# Autodesk Inventor assembly: main
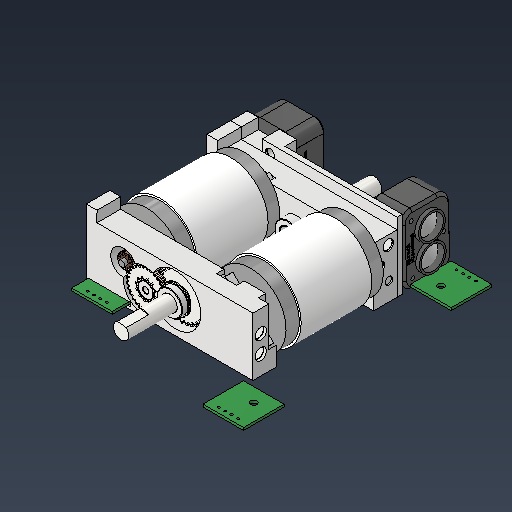
[picture p0: Inventor's stored thumbnail of the model, 512x512]
Saved by Autodesk Inventor 2026.2 (Build 302298010, 298A)
## iProperties
Created: 2026-03-09
Part Number: main
Document SubType Name: Assembly
Designer: szymo
Mass: 365.671 g
Surface Area: 1150.88 cm^2
Volume: 157.658 cm^3
Density: 2.31939 g/cm^3
Author: szymo
## Documents named in this file (18)
- D:\tech\robotyka\robots\evangelion-turbo\inventor-project\main.iam
- D:\tech\robotyka\robots\evangelion-turbo\inventor-project\drive-train.iam
- D:\tech\robotyka\robots\evangelion-turbo\inventor-project\LUNA.ipt
- D:\tech\robotyka\robots\evangelion-turbo\inventor-project\3s450mah.ipt
- D:\tech\robotyka\robots\evangelion-turbo\inventor-project\KTIR-Board.ipt
- D:\tech\robotyka\robots\evangelion-turbo\inventor-project\plug.ipt
- D:\tech\robotyka\robots\evangelion-turbo\inventor-project\FonrtMount.ipt
- D:\tech\robotyka\robots\evangelion-turbo\inventor-project\PCB_interface.ipt
- D:\tech\robotyka\robots\evangelion-turbo\inventor-project\0.96 oled\0.96 oled\0.96 oled.ipt
- D:\tech\robotyka\robots\evangelion-turbo\inventor-project\THMU 13 (SMD JOYSTICK)\THMU 13 (SMD JOYSTICK)\THMU 13 (SMD JOYSTICK).ipt
- D:\tech\robotyka\robots\evangelion-turbo\inventor-project\PCB_Controller.ipt
- D:\tech\robotyka\robots\evangelion-turbo\inventor-project\PCB_Holder_Floor.ipt
- D:\tech\robotyka\robots\evangelion-turbo\inventor-project\SteelFront.ipt
- D:\tech\robotyka\robots\evangelion-turbo\inventor-project\Ceiling.ipt
- D:\tech\robotyka\robots\evangelion-turbo\inventor-project\SpringSteelFront.ipt
- D:\tech\robotyka\robots\evangelion-turbo\inventor-project\LeftGearbox.ipt
- D:\tech\robotyka\robots\evangelion-turbo\inventor-project\LeftGearboxCoverr.ipt
- D:\tech\robotyka\robots\evangelion-turbo\inventor-project\RightGearbox.ipt
## Components (24 placed, 17 different names)
1. drive-train:1 [sub-assembly] — Flush:2, Flush:3, Flush:4, Mate:2, Mate:3, Tangent:1, Mate:18
2. 3s450mah:1 — Flush:8, Tangent:1, Flush:9
3. Ceiling:1 — Flush:64
4. LUNA:2 — Mate:1, Mate:3, Angle:2, Mate:11
5. LUNA:1 — Flush:5, Mate:2, Angle:1, Mate:12
6. LUNA:3 — Flush:22, Flush:23, Mate:6
7. LUNA:4 — Flush:24, Flush:25, Mate:7
8. KTIR-Board:1 — Flush:10, Flush:11, Flush:13
9. KTIR-Board:2 — Mate:4, Flush:12, Flush:14
10. KTIR-Board:4 — Flush:17, Flush:27, Mate:6, Mate:18
11. KTIR-Board:5 — Flush:28, Flush:29, Mate:7, Mate:19
12. SpringSteelFront:1 — Flush:65, Mate:21, Mate:22
13. SteelFront:1 — Flush:62
14. plug:1 — Mate:10, Flush:45, Mate:20
15. FonrtMount:1 — Flush:47
16. PCB_Holder_Floor:1 — Mate:25, Mate:26, Mate:27, Mate:28
17. PCB_Controller:1 — Mate:25, Mate:26
18. PCB_Controller:3 — Mate:27, Mate:28
19. LeftGearbox:1 — Flush:67
20. LeftGearboxCoverr:1 — Flush:69
21. RightGearbox:1 — Flush:71
22. PCB_interface:1 — Mate:14
23. THMU 13 (SMD JOYSTICK):1
24. 0.96 oled:1 — Mate:14
## Relationships (54: Flush 32, Mate 19, Angle 2, Tangent 1)
- Flush:2: drive-train:1
- Flush:3 (-19.2 mm): drive-train:1
- Flush:4: drive-train:1
- Flush:5 (49.5 mm): LUNA:1
- Mate:1 (-49.5 mm): LUNA:2
- Mate:2 (19 mm): drive-train:1 ↔ LUNA:1
- Mate:3 (19 mm): drive-train:1 ↔ LUNA:2
- Angle:1 (-2 deg): LUNA:1
- Angle:2 (182 deg): LUNA:2
- Flush:8 (4.5 mm): 3s450mah:1
- Tangent:1: drive-train:1 ↔ 3s450mah:1
- Flush:9 (-31.5 mm): 3s450mah:1
- Flush:10 (-49 mm): KTIR-Board:1
- Mate:4 (-49 mm): KTIR-Board:2
- Flush:11 (0.13 mm): KTIR-Board:1
- Flush:12 (0.13 mm): KTIR-Board:2
- Flush:13 (66.673 mm): KTIR-Board:1
- Flush:14 (-66.673 mm): KTIR-Board:2
- Flush:17: KTIR-Board:4
- Flush:22: LUNA:3
- Flush:23 (1 mm): LUNA:3
- Flush:24 (1 mm): LUNA:4
- Flush:25: LUNA:4
- Flush:27 (1 mm): KTIR-Board:4
- Flush:28 (1 mm): KTIR-Board:5
- Flush:29: KTIR-Board:5
- Mate:6: LUNA:3 ↔ KTIR-Board:4
- Mate:7: LUNA:4 ↔ KTIR-Board:5
- Mate:10: plug:1
- Flush:45: plug:1
- Mate:11: LUNA:2
- Mate:12: LUNA:1
- Flush:47: FonrtMount:1
- Flush:53 (-29 mm)
- Mate:14: PCB_interface:1 ↔ 0.96 oled:1
- Mate:18: drive-train:1 ↔ KTIR-Board:4
- Mate:19 (19.2 mm): KTIR-Board:5
- Flush:62: SteelFront:1
- Flush:64: Ceiling:1
- Mate:20 (-95.5 mm): plug:1
- Flush:65: SpringSteelFront:1
- Mate:21: SpringSteelFront:1
- Mate:22: SpringSteelFront:1
- Mate:25: PCB_Holder_Floor:1 ↔ PCB_Controller:1
- Mate:26: PCB_Holder_Floor:1 ↔ PCB_Controller:1
- Mate:27: PCB_Holder_Floor:1 ↔ PCB_Controller:3
- Mate:28: PCB_Holder_Floor:1 ↔ PCB_Controller:3
- Flush:66 (-19.2 mm)
- Flush:67: LeftGearbox:1
- Flush:68 (-28.5 mm)
- Flush:69: LeftGearboxCoverr:1
- Flush:70 (19.2 mm)
- Flush:71: RightGearbox:1
- Flush:72 (28.5 mm)
